# Autodesk Inventor assembly: ASY MSC Жабры
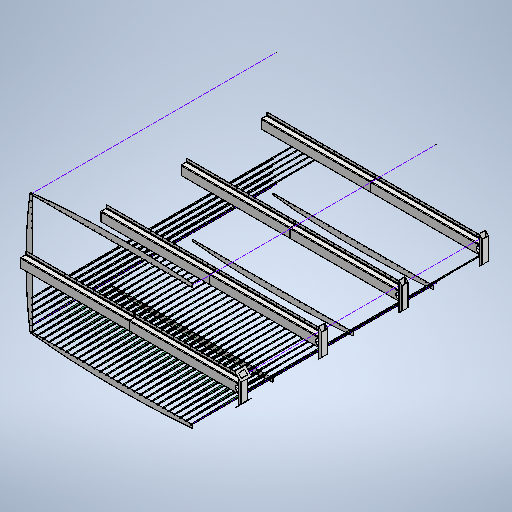
[picture p0: Inventor's stored thumbnail of the model, 512x512]
Saved by Autodesk Inventor 2025 (Build 290162010, 162A)
## iProperties
Created: 2024-08-31
Part Number: ASY MSC Жабры
Document SubType Name: Assembly
Designer: pokla
Author: pokla
## Documents named in this file (22)
- C:\Users\admin\YandexDisk-badmisterfox\домашниий пк\Inventor\Manturovo\Manturovo_Se-clar\ASY MSC Жабры.iam
- C:\Users\admin\YandexDisk-badmisterfox\домашниий пк\Inventor\Manturovo\Manturovo_Se-clar\MSC 0101 sheet gills.ipt
- C:\Users\admin\YandexDisk-badmisterfox\домашниий пк\Inventor\Manturovo\Manturovo_Se-clar\MSC 081 pillar 1.ipt
- C:\Users\admin\YandexDisk-badmisterfox\домашниий пк\Inventor\Manturovo\Manturovo_Se-clar\MSC 0102 sheet gills.ipt
- C:\Users\admin\YandexDisk-badmisterfox\домашниий пк\Inventor\Manturovo\Manturovo_Se-clar\MSC 0202 sheet gills.ipt
- C:\Users\admin\YandexDisk-badmisterfox\домашниий пк\Inventor\Manturovo\Manturovo_Se-clar\MSC 0103 sheet gills.ipt
- C:\Users\admin\YandexDisk-badmisterfox\домашниий пк\Inventor\Manturovo\Manturovo_Se-clar\MSC 0203 sheet gills.ipt
- C:\Users\admin\YandexDisk-badmisterfox\домашниий пк\Inventor\Manturovo\Manturovo_Se-clar\MSC 0104 sheet gills.ipt
- C:\Users\admin\YandexDisk-badmisterfox\домашниий пк\Inventor\Manturovo\Manturovo_Se-clar\MSC 0204 sheet gills.ipt
- C:\Users\admin\YandexDisk-badmisterfox\домашниий пк\Inventor\Manturovo\Manturovo_Se-clar\MSC 0105 sheet gills.ipt
- C:\Users\admin\YandexDisk-badmisterfox\домашниий пк\Inventor\Manturovo\Manturovo_Se-clar\MSC 0205 sheet gills.ipt
- C:\Users\admin\YandexDisk-badmisterfox\домашниий пк\Inventor\Manturovo\Manturovo_Se-clar\MSC 0106 sheet gills.ipt
- C:\Users\admin\YandexDisk-badmisterfox\домашниий пк\Inventor\Manturovo\Manturovo_Se-clar\MSC 0206 sheet gills.ipt
- C:\Users\admin\YandexDisk-badmisterfox\домашниий пк\Inventor\Manturovo\Manturovo_Se-clar\MSC 0107 sheet gills.ipt
- C:\Users\admin\YandexDisk-badmisterfox\домашниий пк\Inventor\Manturovo\Manturovo_Se-clar\MSC 0207 sheet gills.ipt
- C:\Users\admin\YandexDisk-badmisterfox\домашниий пк\Inventor\Manturovo\Manturovo_Se-clar\MSC 079 creen pillar.ipt
- C:\Users\admin\YandexDisk-badmisterfox\домашниий пк\Inventor\Manturovo\Manturovo_Se-clar\MSC DIM 085 tube belly.ipt
- C:\Users\admin\YandexDisk-badmisterfox\домашниий пк\Inventor\Manturovo\Manturovo_Se-clar\MSC 081 pillar 1_CPY.ipt
- C:\Users\admin\YandexDisk-badmisterfox\домашниий пк\Inventor\Manturovo\Manturovo_Se-clar\MSC 0211 string for sheets.ipt
- C:\Users\admin\YandexDisk-badmisterfox\домашниий пк\Inventor\Manturovo\Manturovo_Se-clar\MSC 079 top pillar.ipt
- C:\Users\admin\YandexDisk-badmisterfox\домашниий пк\Inventor\Manturovo\Manturovo_Se-clar\MSC DIM 085.1 heel.ipt
- C:\Users\admin\YandexDisk-badmisterfox\домашниий пк\Inventor\Manturovo\Manturovo_Se-clar\MSC 0201 sheet gills.ipt
## Components (69 placed, 21 different names)
1. MSC DIM 085.1 heel:2 — Rigid:6
2. MSC DIM 085.1 heel:1 — Rigid:7
3. MSC 0102 sheet gills:1 — Rigid:34, Angle:1
4. MSC 0202 sheet gills:1 — Tangent:6, Tangent:7, Rigid:34
5. MSC 0103 sheet gills:1 — Rigid:39
6. MSC 0203 sheet gills:1 — Angle:2, Tangent:8, Tangent:9, Flush:15, Flush:19, Rigid:39
7. MSC 0104 sheet gills:1 — Rigid:36
8. MSC 0204 sheet gills:1 — Rigid:36, Angle:3, Tangent:10, Tangent:11, Flush:15, Flush:16
9. MSC 0105 sheet gills:1 — Rigid:37
10. MSC 0205 sheet gills:1 — Rigid:37, Angle:4, Tangent:12, Tangent:13, Flush:16, Flush:17
11. MSC 0106 sheet gills:1 — Rigid:38
12. MSC 0206 sheet gills:1 — Rigid:38, Angle:5, Tangent:17, Tangent:18, Flush:17, Flush:18
13. MSC 0107 sheet gills:1 — Rigid:32
14. MSC 0207 sheet gills:1 — Rigid:32, Angle:6, Tangent:19, Tangent:20, Flush:18
15. MSC 079 creen pillar:2 — Rigid:15, Rigid:31
16. MSC 079 top pillar:2 — Rigid:24, Rigid:29, Rigid:31
17. MSC 079 top pillar:1 — Rigid:23, Rigid:28, Rigid:30, Tangent:6, Tangent:7, Tangent:8, Tangent:9, Tangent:10, Tangent:11, Tangent:12, Tangent:13, Tangent:17, Tangent:18, Tangent:19, Tangent:20
18. MSC 079 creen pillar:1 — Rigid:12, Rigid:25, Rigid:30, Tangent:14, Tangent:15
19. MSC 0211 string for sheets:2 — Rigid:12
20. MSC 0211 string for sheets:4 — Rigid:15
21. MSC 0211 string for sheets:1 — Rotational:1
22. MSC 0211 string for sheets:3 — Rotational:2
23. MSC 0101 sheet gills.ipt:1 — Rigid:33
24. MSC 0211 string for sheets:143 — Rigid:23
25. MSC 0211 string for sheets:152 — Rigid:24
26. MSC 079 creen pillar:3 — Rigid:25, Rigid:26, Mate:17
27. MSC 079 creen pillar:4 — Rigid:26, Rigid:27
28. MSC 079 creen pillar:5 — Rigid:27
29. MSC DIM 085 tube belly:1 — Rigid:6, Rigid:7, Flush:12, Mate:12, Flush:14, Mate:15, Mate:16, Flush:9
30. MSC 081 pillar 1:1 — Flush:12, Mate:12, Flush:14, Rotational:1, Rotational:2, Tangent:16
31. MSC 081 pillar 1_CPY:1 — Rigid:28, Rigid:29
32. MSC DIM 085 tube belly:2
33. MSC 081 pillar 1:2
34. MSC 081 pillar 1_CPY:2
35. MSC DIM 085 tube belly:3
36. MSC 081 pillar 1:3
37. MSC 081 pillar 1_CPY:3
38. MSC DIM 085 tube belly:4
39. MSC 081 pillar 1:4
40. MSC 081 pillar 1_CPY:4
41. MSC 0201 sheet gills:1 — Mate:17, Rigid:33, Angle:1, Angle:2, Angle:3, Angle:4, Angle:5, Angle:6, Tangent:14, Tangent:15, Tangent:16, Flush:19
42. MSC 0201 sheet gills:2
43. MSC 0201 sheet gills:3
44. MSC 0201 sheet gills:4
45. MSC 0201 sheet gills:5
46. MSC 0201 sheet gills:6
47. MSC 0201 sheet gills:7
48. MSC 0201 sheet gills:8
49. MSC 0201 sheet gills:9
50. MSC 0201 sheet gills:10
51. MSC 0201 sheet gills:11
52. MSC 0201 sheet gills:12
53. MSC 0201 sheet gills:13
54. MSC 0201 sheet gills:14
55. MSC 0201 sheet gills:15
56. MSC 0201 sheet gills:16
57. MSC 0201 sheet gills:17
58. MSC 0201 sheet gills:18
59. MSC 0201 sheet gills:19
60. MSC 0201 sheet gills:20
61. MSC 0201 sheet gills:21
62. MSC 0201 sheet gills:22
63. MSC 0201 sheet gills:23
64. MSC 0201 sheet gills:24
65. MSC 0201 sheet gills:25
66. MSC 0201 sheet gills:26
67. MSC 0201 sheet gills:27
68. MSC 0201 sheet gills:28
69. MSC 0201 sheet gills:29
## Component patterns: (4 elements, first: MSC DIM 085 tube belly:1 + MSC 081 pillar 1:1 + MSC 081 pillar 1_CPY:1), (29 elements, first: MSC 0201 sheet gills:1)
## Relationships (56: WeldJoint 21, Tangent 15, Flush 8, Angle 6, Mate 4, RevoluteJoint 2)
- [WeldJoint]: MSC 081 pillar 1:1 ↔ MSC 081 pillar 1_CPY:1
- Rigid:6 [WeldJoint]: MSC DIM 085.1 heel:2 ↔ MSC DIM 085 tube belly:1
- Rigid:7 [WeldJoint]: MSC DIM 085.1 heel:1 ↔ MSC DIM 085 tube belly:1
- Flush:12: MSC DIM 085 tube belly:1 ↔ MSC 081 pillar 1:1
- Mate:12: MSC DIM 085 tube belly:1 ↔ MSC 081 pillar 1:1
- Flush:14 (5 mm): MSC DIM 085 tube belly:1 ↔ MSC 081 pillar 1:1
- Rigid:12 [WeldJoint] (-5 mm): MSC 079 creen pillar:1 ↔ MSC 0211 string for sheets:2
- Rigid:15 [WeldJoint] (-5 mm): MSC 079 creen pillar:2 ↔ MSC 0211 string for sheets:4
- Mate:15: MSC DIM 085 tube belly:1
- Mate:16: MSC DIM 085 tube belly:1
- Flush:9: MSC DIM 085 tube belly:1
- Rigid:23 [WeldJoint] (-5 mm): MSC 079 top pillar:1 ↔ MSC 0211 string for sheets:143
- Rigid:24 [WeldJoint] (-5 mm): MSC 079 top pillar:2 ↔ MSC 0211 string for sheets:152
- Rigid:25 [WeldJoint] (985 mm): MSC 079 creen pillar:1 ↔ MSC 079 creen pillar:3
- Rigid:26 [WeldJoint] (985 mm): MSC 079 creen pillar:3 ↔ MSC 079 creen pillar:4
- Rigid:27 [WeldJoint] (985 mm): MSC 079 creen pillar:4 ↔ MSC 079 creen pillar:5
- Mate:17: MSC 079 creen pillar:3 ↔ MSC 0201 sheet gills:1
- Rigid:28 [WeldJoint]: MSC 079 top pillar:1 ↔ MSC 081 pillar 1_CPY:1
- Rigid:29 [WeldJoint]: MSC 079 top pillar:2 ↔ MSC 081 pillar 1_CPY:1
- Rigid:30 [WeldJoint]: MSC 079 top pillar:1 ↔ MSC 079 creen pillar:1
- Rigid:31 [WeldJoint]: MSC 079 creen pillar:2 ↔ MSC 079 top pillar:2
- Rotational:1 [RevoluteJoint] (5 mm): MSC 0211 string for sheets:1 ↔ MSC 081 pillar 1:1
- Rotational:2 [RevoluteJoint] (-5 mm): MSC 0211 string for sheets:3 ↔ MSC 081 pillar 1:1
- Tangent:6: MSC 0202 sheet gills:1 ↔ MSC 079 top pillar:1
- Tangent:7: MSC 0202 sheet gills:1 ↔ MSC 079 top pillar:1
- Rigid:32 [WeldJoint]: MSC 0107 sheet gills:1 ↔ MSC 0207 sheet gills:1
- Rigid:33 [WeldJoint] (-10 mm): MSC 0101 sheet gills.ipt:1 ↔ MSC 0201 sheet gills:1
- Rigid:34 [WeldJoint] (-10 mm): MSC 0102 sheet gills:1 ↔ MSC 0202 sheet gills:1
- Rigid:36 [WeldJoint] (-10 mm): MSC 0104 sheet gills:1 ↔ MSC 0204 sheet gills:1
- Rigid:37 [WeldJoint] (-10 mm): MSC 0105 sheet gills:1 ↔ MSC 0205 sheet gills:1
- Rigid:38 [WeldJoint] (-10 mm): MSC 0106 sheet gills:1 ↔ MSC 0206 sheet gills:1
- Angle:1 (0 deg): MSC 0102 sheet gills:1 ↔ MSC 0201 sheet gills:1
- Angle:2 (0 deg): MSC 0203 sheet gills:1 ↔ MSC 0201 sheet gills:1
- Angle:3 (0 deg): MSC 0204 sheet gills:1 ↔ MSC 0201 sheet gills:1
- Angle:4 (0 deg): MSC 0205 sheet gills:1 ↔ MSC 0201 sheet gills:1
- Angle:5 (0 deg): MSC 0206 sheet gills:1 ↔ MSC 0201 sheet gills:1
- Angle:6 (0 deg): MSC 0207 sheet gills:1 ↔ MSC 0201 sheet gills:1
- Tangent:8: MSC 0203 sheet gills:1 ↔ MSC 079 top pillar:1
- Tangent:9: MSC 0203 sheet gills:1 ↔ MSC 079 top pillar:1
- Tangent:10: MSC 0204 sheet gills:1 ↔ MSC 079 top pillar:1
- Tangent:11: MSC 0204 sheet gills:1 ↔ MSC 079 top pillar:1
- Tangent:12: MSC 0205 sheet gills:1 ↔ MSC 079 top pillar:1
- Tangent:13: MSC 0205 sheet gills:1 ↔ MSC 079 top pillar:1
- Tangent:14: MSC 079 creen pillar:1 ↔ MSC 0201 sheet gills:1
- Tangent:15: MSC 079 creen pillar:1 ↔ MSC 0201 sheet gills:1
- Tangent:16: MSC 081 pillar 1:1 ↔ MSC 0201 sheet gills:1
- Tangent:17: MSC 0206 sheet gills:1 ↔ MSC 079 top pillar:1
- Tangent:18: MSC 0206 sheet gills:1 ↔ MSC 079 top pillar:1
- Tangent:19: MSC 0207 sheet gills:1 ↔ MSC 079 top pillar:1
- Tangent:20: MSC 0207 sheet gills:1 ↔ MSC 079 top pillar:1
- Flush:15: MSC 0203 sheet gills:1 ↔ MSC 0204 sheet gills:1
- Flush:16: MSC 0204 sheet gills:1 ↔ MSC 0205 sheet gills:1
- Flush:17: MSC 0205 sheet gills:1 ↔ MSC 0206 sheet gills:1
- Flush:18: MSC 0206 sheet gills:1 ↔ MSC 0207 sheet gills:1
- Flush:19: MSC 0203 sheet gills:1 ↔ MSC 0201 sheet gills:1
- Rigid:39 [WeldJoint] (-10 mm): MSC 0103 sheet gills:1 ↔ MSC 0203 sheet gills:1
